# Autodesk Inventor assembly: Rama_siedziska
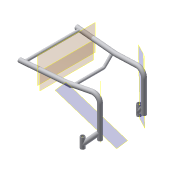
[picture p0: Inventor's stored thumbnail of the model, 180x180]
Saved by Autodesk Inventor 2015 (Build 190159000, 159)
## iProperties
Created: 2015-11-20
Part Number: Rama_siedziska
Document SubType Name: Konstrukcja spawana
Designer: graaapsik
Weld Material: Aluminium AW-7020
Author: graaapsik
## Documents named in this file (7)
- C:\Users\EriveltonDell\Documents\Centro Universitário da FEI\Wheelchair\CADEIRA DE RODAS - DESENHO\Model\Rama_siedziska.iam
- C:\Users\EriveltonDell\Documents\Centro Universitário da FEI\Wheelchair\CADEIRA DE RODAS - DESENHO\Model\Rura_podłużna_ergosiedziska_prawa.ipt
- C:\Users\EriveltonDell\Documents\Centro Universitário da FEI\Wheelchair\CADEIRA DE RODAS - DESENHO\Model\Rura_poprzeczna_ergosiedziska.ipt
- C:\Users\EriveltonDell\Documents\Centro Universitário da FEI\Wheelchair\CADEIRA DE RODAS - DESENHO\Model\Rura_poprzeczna_wygieta.ipt
- C:\Users\EriveltonDell\Documents\Centro Universitário da FEI\Wheelchair\CADEIRA DE RODAS - DESENHO\Model\Rura_podłużna_ergosiedziska_lewa.ipt
- C:\Users\EriveltonDell\Documents\Centro Universitário da FEI\Wheelchair\CADEIRA DE RODAS - DESENHO\Model\Rura_pionowa_kolka_przedniego.ipt
- C:\Users\EriveltonDell\Documents\Centro Universitário da FEI\Wheelchair\CADEIRA DE RODAS - DESENHO\Model\Rura_skosna_kolka_przedniego.ipt
## Components (8 placed, 6 different names)
1. Rura_poprzeczna_ergosiedziska:1 — Równoległy:2, Równoległy:10, Zestawiający:1, Zestawiający:2, Zestawiający:3, Równoległy:11, Styczny:1, Zestawiający:4, Zestawiający:5, Zestawiający:7, Zestawiający:8, Kąt:1
2. Rura_poprzeczna_wygieta:1 — Równoległy:10, Równoległy:12, Równoległy:13
3. Rura_podłużna_ergosiedziska_prawa:1 — Równoległy:2, Zestawiający:1, Zestawiający:2, Równoległy:13, Zestawiający:18, Zestawiający:22
4. Rura_podłużna_ergosiedziska_lewa:1 — Zestawiający:3, Równoległy:11, Styczny:1, Równoległy:12, Zestawiający:10, Zestawiający:16
5. Rura_pionowa_kolka_przedniego:1 — Zestawiający:4, Zestawiający:5, Zestawiający:17, Zestawiający:23, Zestawiający:9
6. Rura_skosna_kolka_przedniego:1 — Zestawiający:21, Zestawiający:22, Zestawiający:23
7. Rura_pionowa_kolka_przedniego:2 — Zestawiający:7, Zestawiający:8, Zestawiający:9, Zestawiający:11, Zestawiający:15
8. Rura_skosna_kolka_przedniego:2 — Zestawiający:14, Zestawiający:15, Zestawiający:16
## Relationships (31: Mate 24, Flush 5, Tangent 1, Angle 1)
- Równoległy:2 [Flush]: Rura_poprzeczna_ergosiedziska:1 ↔ Rura_podłużna_ergosiedziska_prawa:1
- Równoległy:10 [Flush] (270 mm): Rura_poprzeczna_ergosiedziska:1 ↔ Rura_poprzeczna_wygieta:1
- Zestawiający:1 [Mate] (-30 mm): Rura_poprzeczna_ergosiedziska:1 ↔ Rura_podłużna_ergosiedziska_prawa:1
- Zestawiający:2 [Mate] (16 mm): Rura_poprzeczna_ergosiedziska:1 ↔ Rura_podłużna_ergosiedziska_prawa:1
- Zestawiający:3 [Mate] (-30 mm): Rura_poprzeczna_ergosiedziska:1 ↔ Rura_podłużna_ergosiedziska_lewa:1
- Równoległy:11 [Flush]: Rura_poprzeczna_ergosiedziska:1 ↔ Rura_podłużna_ergosiedziska_lewa:1
- Styczny:1 [Tangent]: Rura_poprzeczna_ergosiedziska:1 ↔ Rura_podłużna_ergosiedziska_lewa:1
- Równoległy:12 [Flush] (16 mm): Rura_poprzeczna_wygieta:1 ↔ Rura_podłużna_ergosiedziska_lewa:1
- Równoległy:13 [Flush] (16 mm): Rura_poprzeczna_wygieta:1 ↔ Rura_podłużna_ergosiedziska_prawa:1
- Zestawiający:4 [Mate] (450 mm): Rura_poprzeczna_ergosiedziska:1 ↔ Rura_pionowa_kolka_przedniego:1
- Zestawiający:5 [Mate] (-16 mm): Rura_poprzeczna_ergosiedziska:1 ↔ Rura_pionowa_kolka_przedniego:1
- Zestawiający:7 [Mate] (416 mm): Rura_poprzeczna_ergosiedziska:1 ↔ Rura_pionowa_kolka_przedniego:2
- Zestawiający:8 [Mate] (450 mm): Rura_poprzeczna_ergosiedziska:1 ↔ Rura_pionowa_kolka_przedniego:2
- Zestawiający:9 [Mate]: Rura_pionowa_kolka_przedniego:1 ↔ Rura_pionowa_kolka_przedniego:2
- Zestawiający:10 [Mate]: Rura_podłużna_ergosiedziska_lewa:1
- Zestawiający:11 [Mate]: Rura_pionowa_kolka_przedniego:2
- Zestawiający:12 [Mate]
- Zestawiający:13 [Mate]
- Zestawiający:14 [Mate]: Rura_skosna_kolka_przedniego:2
- Zestawiający:15 [Mate] (16 mm): Rura_pionowa_kolka_przedniego:2 ↔ Rura_skosna_kolka_przedniego:2
- Zestawiający:16 [Mate] (16 mm): Rura_podłużna_ergosiedziska_lewa:1 ↔ Rura_skosna_kolka_przedniego:2
- Zestawiający:17 [Mate]: Rura_pionowa_kolka_przedniego:1
- Zestawiający:18 [Mate]: Rura_podłużna_ergosiedziska_prawa:1
- Zestawiający:19 [Mate]
- Zestawiający:20 [Mate]
- Zestawiający:21 [Mate]: Rura_skosna_kolka_przedniego:1
- Zestawiający:22 [Mate] (16 mm): Rura_podłużna_ergosiedziska_prawa:1 ↔ Rura_skosna_kolka_przedniego:1
- Zestawiający:23 [Mate] (16 mm): Rura_pionowa_kolka_przedniego:1 ↔ Rura_skosna_kolka_przedniego:1
- Kąt:1 [Angle] (0 deg): Rura_poprzeczna_ergosiedziska:1
- Zestawiający:34 [Mate]
- Zestawiający:35 [Mate]
